# Autodesk Inventor assembly: MX-106T+idle.ipt
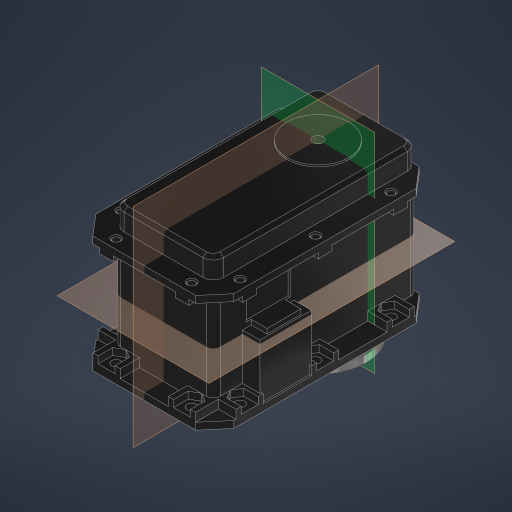
[picture p0: Inventor's stored thumbnail of the model, 512x512]
Saved by Autodesk Inventor 2024 (Build 280153000, 153)
## iProperties
Created: 2022-08-09
Part Number: MX-106T+idle.ipt
Document SubType Name: Assembly
Designer: 박지훈
Author: 박지훈
## Documents named in this file (3)
- C:\Users\ASUS\Desktop\2024_Robit_Hardware\ROBOCUP_2024_eindhoven\부품\ROBOTIS(Inventor 2023 ver.)\다이나믹셀\MX-106T+idle.ipt.iam
- C:\Users\ASUS\Desktop\2024_Robit_Hardware\ROBOCUP_2024_eindhoven\부품\ROBOTIS(Inventor 2023 ver.)\아이들러\64아이들러.iam
- C:\Users\ASUS\Desktop\2024_Robit_Hardware\ROBOCUP_2024_eindhoven\부품\ROBOTIS(Inventor 2023 ver.)\다이나믹셀\MX-106T.ipt
## Components (2 placed, 2 different names)
1. 64아이들러:1 [sub-assembly] — 삽입:1
2. MX-106T:1 — 삽입:1
## Relationships (1: Insert 1)
- 삽입:1 [Insert] (0.06 mm): 64아이들러:1 ↔ MX-106T:1
